# Autodesk Inventor assembly: kowsh
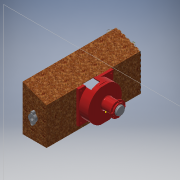
[picture p0: Inventor's stored thumbnail of the model, 180x180]
Saved by Autodesk Inventor 2019 (Build 230136000, 136)
## iProperties
Created: 2022-06-28
Part Number: kowsh
Material: Типовые
Document SubType Name: Assembly
Designer: korsh
Author: korsh
## Documents named in this file (12)
- Z:\Robo\Коршунов Андрей Иванович\36 школа\8 класс\Новая папка (7)\ковш\kowsh.iam
- Z:\Robo\Коршунов Андрей Иванович\36 школа\8 класс\Новая папка (7)\ковш\mot37.ipt
- Z:\Robo\Коршунов Андрей Иванович\36 школа\8 класс\Новая папка (7)\ковш\Двигатель.ipt
- Z:\Robo\Коршунов Андрей Иванович\36 школа\8 класс\Новая папка (7)\ковш\Барабан.ipt
- Z:\Robo\Коршунов Андрей Иванович\36 школа\8 класс\Новая папка (7)\ковш\Лепесток.ipt
- Z:\Robo\Коршунов Андрей Иванович\36 школа\8 класс\Новая папка (7)\ковш\Stenka.ipt
- Z:\Robo\Коршунов Андрей Иванович\36 школа\8 класс\Новая папка (7)\ковш\боковушка.ipt
- Z:\Robo\Коршунов Андрей Иванович\36 школа\8 класс\Новая папка (7)\ковш\верх.ipt
- Z:\Robo\Коршунов Андрей Иванович\36 школа\8 класс\Новая папка (7)\ковш\низ.ipt
- Z:\Robo\Коршунов Андрей Иванович\36 школа\8 класс\Новая папка (7)\ковш\Двигатель червячный.ipt
- Z:\Robo\Коршунов Андрей Иванович\36 школа\8 класс\Новая папка (7)\ковш\боковушка_двиг.ipt
- Z:\Robo\Коршунов Андрей Иванович\36 школа\8 класс\Новая папка (7)\ковш\ппрофиль.ipt
## Components (12 placed, 11 different names)
1. mot37:1 — Совмещение:1, Совмещение:2, Совмещение:3, Заподлицо:4
2. Двигатель:1 — Совмещение:1, Совмещение:3
3. Барабан:1 — Заподлицо:3, Совмещение:2
4. Лепесток:1 — Заподлицо:3
5. Stenka:1 — Заподлицо:4, Заподлицо:5
6. боковушка:1 — Заподлицо:5, Заподлицо:6, Заподлицо:10
7. верх:1 — Заподлицо:7
8. низ:1 — Совмещение:4
9. боковушка_двиг:1 — Совмещение:4, Заподлицо:6, Заподлицо:7, Совмещение:5
10. Двигатель червячный:1 — Совмещение:5, Заподлицо:8, Заподлицо:9
11. Двигатель червячный:2 — Заподлицо:8, Заподлицо:9
12. ппрофиль:1 — Заподлицо:10
## Relationships (13: Flush 8, Mate 5)
- Совмещение:1 [Mate]: mot37:1 ↔ Двигатель:1
- Заподлицо:3 [Flush]: Барабан:1 ↔ Лепесток:1
- Совмещение:2 [Mate]: mot37:1 ↔ Барабан:1
- Совмещение:3 [Mate]: mot37:1 ↔ Двигатель:1
- Заподлицо:4 [Flush]: mot37:1 ↔ Stenka:1
- Заподлицо:5 [Flush]: Stenka:1 ↔ боковушка:1
- Совмещение:4 [Mate]: низ:1 ↔ боковушка_двиг:1
- Заподлицо:6 [Flush]: боковушка:1 ↔ боковушка_двиг:1
- Заподлицо:7 [Flush]: верх:1 ↔ боковушка_двиг:1
- Совмещение:5 [Mate]: боковушка_двиг:1 ↔ Двигатель червячный:1
- Заподлицо:8 [Flush]: Двигатель червячный:1 ↔ Двигатель червячный:2
- Заподлицо:9 [Flush]: Двигатель червячный:1 ↔ Двигатель червячный:2
- Заподлицо:10 [Flush]: боковушка:1 ↔ ппрофиль:1
